# Autodesk Inventor assembly: e3d v6
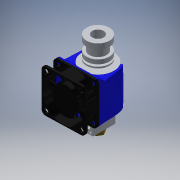
[picture p0: Inventor's stored thumbnail of the model, 180x180]
Saved by Autodesk Inventor 2019 (Build 230136000, 136)
## iProperties
Created: 2017-12-19
Part Number: e3d v6
Description: STEP AP214
Document SubType Name: Assembly
Designer: rah75
Sending System: SolidWorks 2016
Preprocessor: SwSTEP 2.0
Title: e3d v6.STEP
Revision Number: ANY
## Documents named in this file (6)
- C:\Users\rah75\Box\CAD\3D Printer\e3d-v6-hotend-3\e3d v6.iam
- C:\Users\rah75\Box\CAD\3D Printer\e3d-v6-hotend-3\e3d nozzle (0.4).ipt
- C:\Users\rah75\Box\CAD\3D Printer\e3d-v6-hotend-3\e3d heaterblock.ipt
- C:\Users\rah75\Box\CAD\3D Printer\e3d-v6-hotend-3\e3d heat break.ipt
- C:\Users\rah75\Box\CAD\3D Printer\e3d-v6-hotend-3\e3d heatsink.ipt
- C:\Users\rah75\Box\CAD\3D Printer\e3d-v6-hotend-3\fanduct.iam
## Components (5 placed, 5 different names)
1. e3d nozzle (0.4)_1
2. e3d heaterblock_2
3. e3d heat break_3
4. e3d heatsink_4 — Insert:1
5. fanduct_5 [sub-assembly] — Insert:1
## Relationships (1: Insert 1)
- Insert:1: e3d heatsink_4 ↔ fanduct_5
